# Autodesk Inventor assembly: Base Fall 2014
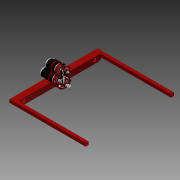
[picture p0: Inventor's stored thumbnail of the model, 180x180]
Saved by Autodesk Inventor 2013 (Build 170138000, 138)
## iProperties
Created: 2013-06-29
Part Number: Base Fall 2014
Document SubType Name: Assembly
Designer: mvarma
Author: mvarma
## Documents named in this file (5)
- C:\Users\mvarma\Desktop\GRT 2013-2014 Gearbox\Base\Base Fall 2014.iam
- C:\Users\mvarma\Desktop\GRT 2013-2014 Gearbox\Base\Box Beam\Front Support.ipt
- C:\Users\mvarma\Desktop\GRT 2013-2014 Gearbox\Base\Box Beam\Rear Support.ipt
- C:\Users\mvarma\Desktop\GRT 2013-2014 Gearbox\Base\Box Beam\Tube - Left.ipt
- C:\Users\mvarma\Desktop\GRT 2013-2014 Gearbox\Mark 4\Mark 4.5.iam
## Components (4 placed, 4 different names)
1. Tube - Left:1 — Mate:1, Mate:2, Mate:3, Mate:4, Mate:5, Mate:6, Mate:7, Mate:8, Mate:9
2. Front Support:1 — Mate:1, Mate:2, Mate:3
3. Rear Support:1 — Mate:4, Mate:5, Mate:6
4. Mark 4.5:1 [sub-assembly] — Mate:7, Mate:8, Mate:9
## Relationships (9: Mate 9)
- Mate:1: Tube - Left:1 ↔ Front Support:1
- Mate:2: Tube - Left:1 ↔ Front Support:1
- Mate:3: Tube - Left:1 ↔ Front Support:1
- Mate:4: Tube - Left:1 ↔ Rear Support:1
- Mate:5: Tube - Left:1 ↔ Rear Support:1
- Mate:6: Tube - Left:1 ↔ Rear Support:1
- Mate:7: Tube - Left:1 ↔ Mark 4.5:1
- Mate:8: Tube - Left:1 ↔ Mark 4.5:1
- Mate:9: Tube - Left:1 ↔ Mark 4.5:1
